# Autodesk Inventor assembly: Assemblylatest
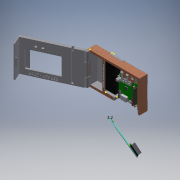
[picture p0: Inventor's stored thumbnail of the model, 180x180]
Saved by Autodesk Inventor 2017 (Build 210142000, 142)
## iProperties
Created: 2016-12-22
Part Number: Assemblylatest
Document SubType Name: Assembly
Designer: radrajith
Author: radrajith
## Documents named in this file (8)
- C:\Users\radra\Box Sync\Senior Fall 2016\ESE 323\autocad\Assemblylatest.iam
- C:\Users\radra\Box Sync\Senior Fall 2016\ESE 323\autocad\case_bottom.ipt
- C:\Users\radra\Box Sync\Senior Fall 2016\ESE 323\autocad\battery_cover.ipt
- C:\Users\radra\Box Sync\Senior Fall 2016\ESE 323\autocad\case top_new.ipt
- C:\Users\radra\Box Sync\Senior Fall 2016\ESE 323\autocad\lab 04.ipt
- C:\Users\radra\Box Sync\Senior Fall 2016\ESE 323\autocad\battery.ipt
- C:\Users\radra\Box Sync\Senior Fall 2016\ESE 323\autocad\button_press_new.ipt
- C:\Users\radra\Box Sync\Senior Fall 2016\ESE 323\autocad\lcd display.ipt
## Components (8 placed, 7 different names)
1. case_bottom:1 — Mate:1, Mate:2, Mate:3, Mate:4, Mate:5, Mate:8, Mate:10
2. battery_cover:1 — Mate:1, Mate:2, Mate:3, Mate:9
3. case top_new:1 — Mate:4, Mate:5
4. lab 04:1 — Mate:8, Mate:12, Mate:13
5. battery:1 — Mate:9, Mate:10
6. button_press_new:1 — Mate:12
7. button_press_new:2 — Mate:13
8. lcd display:1
## Relationships (10: Mate 10)
- Mate:1: case_bottom:1 ↔ battery_cover:1
- Mate:2: case_bottom:1 ↔ battery_cover:1
- Mate:3 (2.929 mm): case_bottom:1 ↔ battery_cover:1
- Mate:4: case_bottom:1 ↔ case top_new:1
- Mate:5 (0.5 mm): case_bottom:1 ↔ case top_new:1
- Mate:8 (2 mm): case_bottom:1 ↔ lab 04:1
- Mate:9: battery_cover:1 ↔ battery:1
- Mate:10: case_bottom:1 ↔ battery:1
- Mate:12 (1 mm): lab 04:1 ↔ button_press_new:1
- Mate:13 (1 mm): lab 04:1 ↔ button_press_new:2
